# Autodesk Inventor assembly: Behavioural Device assembly 2
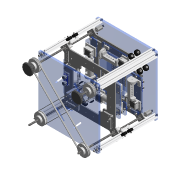
[picture p0: Inventor's stored thumbnail of the model, 180x180]
Saved by Autodesk Inventor 2020 (Build 240168000, 168)
## iProperties
Created: 2020-08-17
Part Number: Behavioural Device assembly 2
Document SubType Name: Assembly
Designer: ferrerx
Author: ferrerx
## Documents named in this file (17)
- C:\Users\ferrerx\Desktop\Projects\Prieto-Godino Lab\Drosophila Larvae Behavioural Device\Device design V3\Inventor Assembly\Behavioural Device assembly 2.iam
- C:\Users\ferrerx\Desktop\Projects\Prieto-Godino Lab\Drosophila Larvae Behavioural Device\Device design V3\Inventor Assembly\aluminum profile.ipt
- C:\Users\ferrerx\Desktop\Projects\Prieto-Godino Lab\Drosophila Larvae Behavioural Device\Device design V3\Inventor Assembly\Z stage Base.ipt
- C:\Users\ferrerx\Desktop\Projects\Prieto-Godino Lab\Drosophila Larvae Behavioural Device\Device design V3\Inventor Assembly\Big pulley.ipt
- C:\Users\ferrerx\Desktop\Projects\Prieto-Godino Lab\Drosophila Larvae Behavioural Device\Device design V3\Inventor Assembly\Shaft connector.ipt
- C:\Users\ferrerx\Desktop\Projects\Prieto-Godino Lab\Drosophila Larvae Behavioural Device\Device design V3\Inventor Assembly\Lead screw.ipt
- C:\Users\ferrerx\Desktop\Projects\Prieto-Godino Lab\Drosophila Larvae Behavioural Device\Device design V3\Inventor Assembly\Lead screw manual adjuster.ipt
- C:\Users\ferrerx\Desktop\Projects\Prieto-Godino Lab\Drosophila Larvae Behavioural Device\Device design V3\Inventor Assembly\Z stage Roof 2.ipt
- C:\Users\ferrerx\Desktop\Projects\Prieto-Godino Lab\Drosophila Larvae Behavioural Device\Device design V3\Inventor Assembly\Belt.ipt
- C:\Users\ferrerx\Documents\Inventor\Content Center Files\R2020\en-US\AS 1427(10)\AS 1427 - M5 x 16(7).ipt
- C:\Users\ferrerx\Documents\Inventor\Content Center Files\R2020\en-US\AS 1427(10)\AS 1427 - M4 x 16(7).ipt
- C:\Users\ferrerx\Desktop\Projects\Prieto-Godino Lab\Drosophila Larvae Behavioural Device\Device design V3\Inventor Assembly\Arena assembly.iam
- C:\Users\ferrerx\Desktop\Projects\Prieto-Godino Lab\Drosophila Larvae Behavioural Device\Device design V3\Inventor Assembly\Linear actuator assem 1.iam
- C:\Users\ferrerx\Desktop\Projects\Prieto-Godino Lab\Drosophila Larvae Behavioural Device\Device design V3\Inventor Assembly\Platform assembly with IR.iam
- C:\Users\ferrerx\Desktop\Projects\Prieto-Godino Lab\Drosophila Larvae Behavioural Device\Device design V3\Inventor Assembly\Platform RGB assembly.iam
- C:\Users\ferrerx\Documents\Inventor\Content Center Files\R2020\en-US\AS 1427(10)\AS 1427 - M3 x 16(7).ipt
- C:\Users\ferrerx\Documents\Inventor\Content Center Files\R2020\en-US\AS 1427(10)\AS 1427 - M5 x 12(7).ipt
## Components (58 placed, 16 different names)
1. aluminum profile:1 — Mate:7, Mate:8, Mate:9, Mate:102, Mate:103, Mate:104
2. aluminum profile:2 — Mate:1, Mate:2, Mate:3, Angle:1
3. Z stage Base:2 — Mate:1, Mate:2, Mate:3, Mate:4, Mate:5, Mate:6, Mate:7, Mate:8, Mate:9, Mate:10, Mate:11, Mate:12, Mate:75, Mate:76, Mate:77, Mate:78, Mate:145, Mate:146, Mate:147, Mate:148, Mate:276, Mate:277, Mate:278, Mate:279, Mate:282, Mate:283, Mate:284, Mate:285, Mate:292, Mate:293, Mate:294, Mate:295, Mate:298, Mate:299, Mate:300, Mate:301, Mate:312, Mate:313, Mate:314, Mate:315, Mate:316, Mate:317, Mate:318, Mate:319, Mate:328, Mate:338, Mate:339, Mate:340, Mate:341
4. aluminum profile:3 — Mate:10, Mate:11, Mate:12
5. aluminum profile:4 — Mate:4, Mate:5, Mate:6, Angle:2
6. Big pulley:1 — Mate:95, Mate:106, Mate:325
7. Big pulley:2 — Mate:94, Mate:105, Mate:251, Mate:252, Mate:321
8. Shaft connector:1 — Mate:75, Mate:76, Mate:79, Mate:81
9. Shaft connector:2 — Mate:77, Mate:78, Mate:82, Mate:83
10. Lead screw:3 — Mate:79, Mate:81, Mate:94, Mate:99, Mate:100, Mate:336
11. Lead screw:4 — Mate:82, Mate:83, Mate:95
12. Lead screw manual adjuster:2 — Mate:99, Mate:100, Mate:320
13. Z stage Roof 2:1 — Mate:102, Mate:103, Mate:104, Mate:105, Mate:106, Mate:272, Mate:273, Mate:274, Mate:275, Mate:280, Mate:281, Mate:286, Mate:287, Mate:288, Mate:289, Mate:290, Mate:291, Mate:296, Mate:297, Mate:302, Mate:303, Mate:329, Mate:330, Mate:331, Mate:332, Mate:333, Mate:334, Mate:335
14. Lead screw:5 — Mate:149, Mate:151, Mate:154, Mate:156, Mate:157
15. Lead screw:6 — Mate:150, Mate:152, Mate:153, Mate:337
16. Lead screw manual adjuster:3 — Mate:156, Mate:157, Mate:160, Mate:323
17. Big pulley:3 — Mate:154, Mate:160, Mate:253, Mate:254, Mate:322
18. Big pulley:4 — Mate:153, Mate:324
19. Shaft connector:3 — Mate:145, Mate:148, Mate:150, Mate:152
20. Shaft connector:4 — Mate:146, Mate:147, Mate:149, Mate:151
21. Belt:1 — Mate:251, Mate:252
22. Belt:2 — Mate:253, Mate:254
23. AS 1427 (8) - Metric M5 x 16:1 — Mate:273, Mate:275
24. AS 1427 (8) - Metric M5 x 16:2 — Mate:277, Mate:279
25. AS 1427 (8) - Metric M5 x 16:3 — Mate:272, Mate:274
26. AS 1427 (8) - Metric M5 x 16:4 — Mate:280, Mate:286
27. AS 1427 (8) - Metric M5 x 16:5 — Mate:283, Mate:284
28. AS 1427 (8) - Metric M5 x 16:6 — Mate:288, Mate:290
29. AS 1427 (8) - Metric M5 x 16:7 — Mate:281, Mate:287
30. AS 1427 (8) - Metric M5 x 16:8 — Mate:282, Mate:285
31. AS 1427 (8) - Metric M5 x 16:9 — Mate:293, Mate:295
32. AS 1427 (8) - Metric M5 x 16:10 — Mate:289, Mate:291
33. AS 1427 (8) - Metric M5 x 16:11 — Mate:298, Mate:301
34. AS 1427 (8) - Metric M5 x 16:12 — Mate:296, Mate:303
35. AS 1427 (8) - Metric M5 x 16:13 — Mate:299, Mate:300
36. AS 1427 (8) - Metric M5 x 16:14 — Mate:276, Mate:278
37. AS 1427 (8) - Metric M5 x 16:15 — Mate:292, Mate:294
38. AS 1427 (8) - Metric M5 x 16:16 — Mate:297, Mate:302
39. AS 1427 (8) - Metric M4 x 16:1 — Mate:322
40. AS 1427 (8) - Metric M4 x 16:2 — Mate:320
41. AS 1427 (8) - Metric M4 x 16:3 — Mate:313, Mate:319
42. AS 1427 (8) - Metric M4 x 16:4 — Mate:321
43. AS 1427 (8) - Metric M4 x 16:5 — Mate:314, Mate:318, Mate:327
44. AS 1427 (8) - Metric M4 x 16:6 — Mate:315, Mate:316, Mate:326
45. AS 1427 (8) - Metric M4 x 16:7 — Mate:323
46. AS 1427 (8) - Metric M4 x 16:8 — Mate:312, Mate:317
47. AS 1427 (8) - Metric M4 x 16:9 — Mate:324
48. AS 1427 (8) - Metric M4 x 16:10 — Mate:325
49. Arena assembly:1 [sub-assembly] — Mate:326, Mate:327, Mate:328
50. Linear actuator assem 1:1 [sub-assembly] — Mate:329, Mate:330, Mate:331
51. Platform assembly with IR:1 [sub-assembly] — Mate:336, Angle:1
52. Platform RGB assembly:1 [sub-assembly] — Mate:337, Angle:2
53. AS 1427 (8) - Metric M3 x 16:1 — Mate:332, Mate:334
54. AS 1427 (8) - Metric M3 x 16:2 — Mate:333, Mate:335
55. AS 1427 (8) - Metric M5 x 12:1 — Mate:338
56. AS 1427 (8) - Metric M5 x 12:2 — Mate:339
57. AS 1427 (8) - Metric M5 x 12:3 — Mate:341
58. AS 1427 (8) - Metric M5 x 12:4 — Mate:340
## Relationships (110: Mate 108, Angle 2)
- Mate:1: aluminum profile:2 ↔ Z stage Base:2
- Mate:2: aluminum profile:2 ↔ Z stage Base:2
- Mate:3: aluminum profile:2 ↔ Z stage Base:2
- Mate:4: Z stage Base:2 ↔ aluminum profile:4
- Mate:5: Z stage Base:2 ↔ aluminum profile:4
- Mate:6: Z stage Base:2 ↔ aluminum profile:4
- Mate:7: aluminum profile:1 ↔ Z stage Base:2
- Mate:8: aluminum profile:1 ↔ Z stage Base:2
- Mate:9: aluminum profile:1 ↔ Z stage Base:2
- Mate:10: Z stage Base:2 ↔ aluminum profile:3
- Mate:11: Z stage Base:2 ↔ aluminum profile:3
- Mate:12: Z stage Base:2 ↔ aluminum profile:3
- Mate:75: Z stage Base:2 ↔ Shaft connector:1
- Mate:76: Z stage Base:2 ↔ Shaft connector:1
- Mate:77: Z stage Base:2 ↔ Shaft connector:2
- Mate:78: Z stage Base:2 ↔ Shaft connector:2
- Mate:79: Shaft connector:1 ↔ Lead screw:3
- Mate:81: Shaft connector:1 ↔ Lead screw:3
- Mate:82: Shaft connector:2 ↔ Lead screw:4
- Mate:83: Shaft connector:2 ↔ Lead screw:4
- Mate:94: Big pulley:2 ↔ Lead screw:3
- Mate:95: Big pulley:1 ↔ Lead screw:4
- Mate:99: Lead screw:3 ↔ Lead screw manual adjuster:2
- Mate:100: Lead screw:3 ↔ Lead screw manual adjuster:2
- Mate:102: aluminum profile:1 ↔ Z stage Roof 2:1
- Mate:103: aluminum profile:1 ↔ Z stage Roof 2:1
- Mate:104: aluminum profile:1 ↔ Z stage Roof 2:1
- Mate:105: Big pulley:2 ↔ Z stage Roof 2:1
- Mate:106: Big pulley:1 ↔ Z stage Roof 2:1
- Mate:145: Z stage Base:2 ↔ Shaft connector:3
- Mate:146: Z stage Base:2 ↔ Shaft connector:4
- Mate:147: Z stage Base:2 ↔ Shaft connector:4
- Mate:148: Z stage Base:2 ↔ Shaft connector:3
- Mate:149: Lead screw:5 ↔ Shaft connector:4
- Mate:150: Lead screw:6 ↔ Shaft connector:3
- Mate:151: Lead screw:5 ↔ Shaft connector:4
- Mate:152: Lead screw:6 ↔ Shaft connector:3
- Mate:153: Lead screw:6 ↔ Big pulley:4
- Mate:154: Lead screw:5 ↔ Big pulley:3
- Mate:156: Lead screw:5 ↔ Lead screw manual adjuster:3
- Mate:157: Lead screw:5 ↔ Lead screw manual adjuster:3
- Mate:160: Lead screw manual adjuster:3 ↔ Big pulley:3
- Mate:251: Big pulley:2 ↔ Belt:1
- Mate:252 (1 mm): Big pulley:2 ↔ Belt:1
- Mate:253: Big pulley:3 ↔ Belt:2
- Mate:254 (1 mm): Big pulley:3 ↔ Belt:2
- Mate:272: Z stage Roof 2:1 ↔ AS 1427 (8) - Metric M5 x 16:3
- Mate:273: Z stage Roof 2:1 ↔ AS 1427 (8) - Metric M5 x 16:1
- Mate:274: Z stage Roof 2:1 ↔ AS 1427 (8) - Metric M5 x 16:3
- Mate:275: Z stage Roof 2:1 ↔ AS 1427 (8) - Metric M5 x 16:1
- Mate:276: Z stage Base:2 ↔ AS 1427 (8) - Metric M5 x 16:14
- Mate:277: Z stage Base:2 ↔ AS 1427 (8) - Metric M5 x 16:2
- Mate:278: Z stage Base:2 ↔ AS 1427 (8) - Metric M5 x 16:14
- Mate:279: Z stage Base:2 ↔ AS 1427 (8) - Metric M5 x 16:2
- Mate:280: Z stage Roof 2:1 ↔ AS 1427 (8) - Metric M5 x 16:4
- Mate:281: Z stage Roof 2:1 ↔ AS 1427 (8) - Metric M5 x 16:7
- Mate:282: Z stage Base:2 ↔ AS 1427 (8) - Metric M5 x 16:8
- Mate:283: Z stage Base:2 ↔ AS 1427 (8) - Metric M5 x 16:5
- Mate:284: Z stage Base:2 ↔ AS 1427 (8) - Metric M5 x 16:5
- Mate:285: Z stage Base:2 ↔ AS 1427 (8) - Metric M5 x 16:8
- Mate:286: Z stage Roof 2:1 ↔ AS 1427 (8) - Metric M5 x 16:4
- Mate:287: Z stage Roof 2:1 ↔ AS 1427 (8) - Metric M5 x 16:7
- Mate:288: Z stage Roof 2:1 ↔ AS 1427 (8) - Metric M5 x 16:6
- Mate:289: Z stage Roof 2:1 ↔ AS 1427 (8) - Metric M5 x 16:10
- Mate:290: Z stage Roof 2:1 ↔ AS 1427 (8) - Metric M5 x 16:6
- Mate:291: Z stage Roof 2:1 ↔ AS 1427 (8) - Metric M5 x 16:10
- Mate:292: Z stage Base:2 ↔ AS 1427 (8) - Metric M5 x 16:15
- Mate:293: Z stage Base:2 ↔ AS 1427 (8) - Metric M5 x 16:9
- Mate:294: Z stage Base:2 ↔ AS 1427 (8) - Metric M5 x 16:15
- Mate:295: Z stage Base:2 ↔ AS 1427 (8) - Metric M5 x 16:9
- Mate:296: Z stage Roof 2:1 ↔ AS 1427 (8) - Metric M5 x 16:12
- Mate:297: Z stage Roof 2:1 ↔ AS 1427 (8) - Metric M5 x 16:16
- Mate:298: Z stage Base:2 ↔ AS 1427 (8) - Metric M5 x 16:11
- Mate:299: Z stage Base:2 ↔ AS 1427 (8) - Metric M5 x 16:13
- Mate:300: Z stage Base:2 ↔ AS 1427 (8) - Metric M5 x 16:13
- Mate:301: Z stage Base:2 ↔ AS 1427 (8) - Metric M5 x 16:11
- Mate:302: Z stage Roof 2:1 ↔ AS 1427 (8) - Metric M5 x 16:16
- Mate:303: Z stage Roof 2:1 ↔ AS 1427 (8) - Metric M5 x 16:12
- Mate:312: Z stage Base:2 ↔ AS 1427 (8) - Metric M4 x 16:8
- Mate:313: Z stage Base:2 ↔ AS 1427 (8) - Metric M4 x 16:3
- Mate:314: Z stage Base:2 ↔ AS 1427 (8) - Metric M4 x 16:5
- Mate:315: Z stage Base:2 ↔ AS 1427 (8) - Metric M4 x 16:6
- Mate:316: Z stage Base:2 ↔ AS 1427 (8) - Metric M4 x 16:6
- Mate:317: Z stage Base:2 ↔ AS 1427 (8) - Metric M4 x 16:8
- Mate:318: Z stage Base:2 ↔ AS 1427 (8) - Metric M4 x 16:5
- Mate:319: Z stage Base:2 ↔ AS 1427 (8) - Metric M4 x 16:3
- Mate:320: Lead screw manual adjuster:2 ↔ AS 1427 (8) - Metric M4 x 16:2
- Mate:321: Big pulley:2 ↔ AS 1427 (8) - Metric M4 x 16:4
- Mate:322: Big pulley:3 ↔ AS 1427 (8) - Metric M4 x 16:1
- Mate:323: Lead screw manual adjuster:3 ↔ AS 1427 (8) - Metric M4 x 16:7
- Mate:324: Big pulley:4 ↔ AS 1427 (8) - Metric M4 x 16:9
- Mate:325: Big pulley:1 ↔ AS 1427 (8) - Metric M4 x 16:10
- Mate:326: AS 1427 (8) - Metric M4 x 16:6 ↔ Arena assembly:1
- Mate:327: AS 1427 (8) - Metric M4 x 16:5 ↔ Arena assembly:1
- Mate:328: Z stage Base:2 ↔ Arena assembly:1
- Mate:329: Z stage Roof 2:1 ↔ Linear actuator assem 1:1
- Mate:330: Z stage Roof 2:1 ↔ Linear actuator assem 1:1
- Mate:331: Z stage Roof 2:1 ↔ Linear actuator assem 1:1
- Mate:332: Z stage Roof 2:1 ↔ AS 1427 (8) - Metric M3 x 16:1
- Mate:333: Z stage Roof 2:1 ↔ AS 1427 (8) - Metric M3 x 16:2
- Mate:334: Z stage Roof 2:1 ↔ AS 1427 (8) - Metric M3 x 16:1
- Mate:335: Z stage Roof 2:1 ↔ AS 1427 (8) - Metric M3 x 16:2
- Mate:336: Lead screw:3 ↔ Platform assembly with IR:1
- Angle:1 (0 deg): aluminum profile:2 ↔ Platform assembly with IR:1
- Mate:337: Lead screw:6 ↔ Platform RGB assembly:1
- Angle:2 (0 deg): aluminum profile:4 ↔ Platform RGB assembly:1
- Mate:338: Z stage Base:2 ↔ AS 1427 (8) - Metric M5 x 12:1
- Mate:339: Z stage Base:2 ↔ AS 1427 (8) - Metric M5 x 12:2
- Mate:340: Z stage Base:2 ↔ AS 1427 (8) - Metric M5 x 12:4
- Mate:341: Z stage Base:2 ↔ AS 1427 (8) - Metric M5 x 12:3
